# Autodesk Inventor assembly: Foot-40x
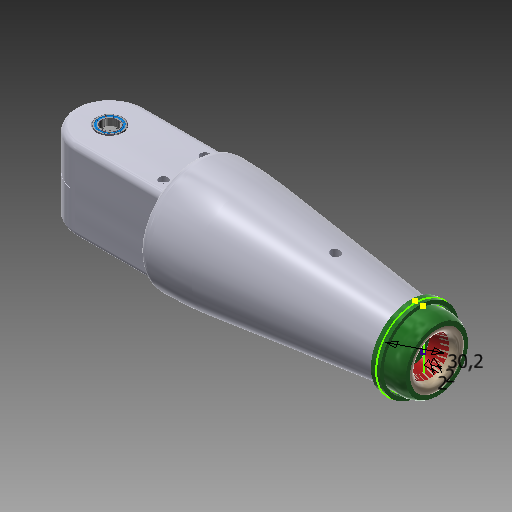
[picture p0: Inventor's stored thumbnail of the model, 512x512]
Saved by Autodesk Inventor 2018 (Build 220112000, 112)
## iProperties
Created: 2017-08-24
Part Number: Foot-40x
Material: Generisch
Document SubType Name: Assembly
Designer: JochenAlt
Author: JochenAlt
## Documents named in this file (4)
- D:\Projects\Manfred\design\cad\Inventor\Foot-40x.iam
- D:\Projects\Manfred\design\cad\Inventor\Foot-40x.ipt
- D:\Projects\Manfred\design\cad\Inventor\Rillenkugellager 11x7x3 inafag smr117.ipt
- D:\Projects\Manfred\design\cad\Inventor\Herkulex DRS-010x\HerkuleX DRS-0101.iam
## Components (3 placed, 3 different names)
1. Foot-40x:1 — Passend:1, Passend:2, Passend:3, Passend:4
2. Rillenkugellager 11x7x3 inafag smr117:1 — Passend:4, Passend:5
3. HerkuleX DRS-0101:1 [sub-assembly] — Passend:1, Passend:2, Passend:3, Passend:5
## Relationships (5: Mate 5)
- Passend:1 [Mate]: Foot-40x:1 ↔ HerkuleX DRS-0101:1
- Passend:2 [Mate]: Foot-40x:1 ↔ HerkuleX DRS-0101:1
- Passend:3 [Mate]: Foot-40x:1 ↔ HerkuleX DRS-0101:1
- Passend:4 [Mate]: Foot-40x:1 ↔ Rillenkugellager 11x7x3 inafag smr117:1
- Passend:5 [Mate]: Rillenkugellager 11x7x3 inafag smr117:1 ↔ HerkuleX DRS-0101:1
